# Autodesk Inventor assembly: Assembly1
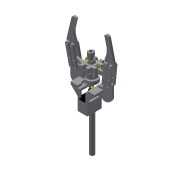
[picture p0: Inventor's stored thumbnail of the model, 180x180]
Saved by Autodesk Inventor 2018 (Build 220112000, 112)
## iProperties
Created: 2018-02-12
Part Number: Assembly1
Document SubType Name: Assembly
Designer: Bardo91
Author: Bardo91
## Documents named in this file (9)
- E:\programming\hecatonquiros\cad_models\tools\gripper\serial_model\Assembly1.iam
- E:\programming\hecatonquiros\cad_models\tools\gripper\serial_model\core_structure.ipt
- E:\programming\hecatonquiros\cad_models\tools\gripper\serial_model\holdBar.ipt
- E:\programming\hecatonquiros\cad_models\tools\gripper\serial_model\ScrewActuatorGripper.ipt
- E:\programming\hecatonquiros\cad_models\tools\gripper\serial_model\microservo_FT.ipt
- E:\programming\hecatonquiros\cad_models\tools\gripper\serial_model\bar.ipt
- E:\programming\hecatonquiros\cad_models\tools\gripper\serial_model\gripper.ipt
- E:\programming\hecatonquiros\cad_models\tools\gripper\serial_model\ScrewActuatorGripperCenter.ipt
- E:\programming\hecatonquiros\cad_models\tools\gripper\serial_model\barMini.ipt
## Components (18 placed, 8 different names)
1. core_structure:1 — Mate:1, Mate:2, Mate:3, Mate:4, Mate:5, Mate:6, Mate:7, Mate:8, Mate:9, Mate:10
2. holdBar:1 — Mate:4, Mate:5, Mate:6, Mate:11, Mate:12, Mate:13, Mate:14, Mate:15, Mate:16, Mate:17, Mate:18
3. holdBar:2 — Mate:1, Mate:2, Mate:3, Mate:19, Mate:20, Mate:21, Mate:22, Mate:23, Mate:24, Mate:25, Mate:26
4. ScrewActuatorGripper:1 — Mate:7, Mate:37, Mate:38
5. microservo_FT:1 — Mate:8, Mate:9, Mate:10
6. bar:1 — Mate:11, Mate:12, Mate:31
7. bar:2 — Mate:13, Mate:14, Mate:30, Mate:40
8. bar:3 — Mate:15, Mate:18, Mate:27, Mate:28
9. bar:4 — Mate:16, Mate:17, Mate:29
10. bar:5 — Mate:19, Mate:21, Mate:34, Mate:42
11. bar:6 — Mate:20, Mate:22, Mate:32, Mate:33
12. bar:7 — Mate:23, Mate:26, Mate:35
13. bar:8 — Mate:24, Mate:25, Mate:36
14. gripper:1 — Mate:27, Mate:28, Mate:29, Mate:30, Mate:31
15. gripper:2 — Mate:32, Mate:33, Mate:34, Mate:35, Mate:36
16. ScrewActuatorGripperCenter:1 — Mate:37, Mate:38, Mate:39, Mate:41, Mate:43, Mate:44
17. barMini:1 — Mate:39, Mate:40, Mate:41
18. barMini:2 — Mate:42, Mate:43, Mate:44
## Relationships (44: Mate 44)
- Mate:1: core_structure:1 ↔ holdBar:2
- Mate:2: core_structure:1 ↔ holdBar:2
- Mate:3: core_structure:1 ↔ holdBar:2
- Mate:4: core_structure:1 ↔ holdBar:1
- Mate:5: core_structure:1 ↔ holdBar:1
- Mate:6: core_structure:1 ↔ holdBar:1
- Mate:7: core_structure:1 ↔ ScrewActuatorGripper:1
- Mate:8: core_structure:1 ↔ microservo_FT:1
- Mate:9: core_structure:1 ↔ microservo_FT:1
- Mate:10: core_structure:1 ↔ microservo_FT:1
- Mate:11: holdBar:1 ↔ bar:1
- Mate:12: holdBar:1 ↔ bar:1
- Mate:13: holdBar:1 ↔ bar:2
- Mate:14: holdBar:1 ↔ bar:2
- Mate:15: holdBar:1 ↔ bar:3
- Mate:16: holdBar:1 ↔ bar:4
- Mate:17: holdBar:1 ↔ bar:4
- Mate:18: holdBar:1 ↔ bar:3
- Mate:19: holdBar:2 ↔ bar:5
- Mate:20: holdBar:2 ↔ bar:6
- Mate:21: holdBar:2 ↔ bar:5
- Mate:22: holdBar:2 ↔ bar:6
- Mate:23: holdBar:2 ↔ bar:7
- Mate:24: holdBar:2 ↔ bar:8
- Mate:25: holdBar:2 ↔ bar:8
- Mate:26: holdBar:2 ↔ bar:7
- Mate:27: bar:3 ↔ gripper:1
- Mate:28: bar:3 ↔ gripper:1
- Mate:29: bar:4 ↔ gripper:1
- Mate:30: bar:2 ↔ gripper:1
- Mate:31: bar:1 ↔ gripper:1
- Mate:32: bar:6 ↔ gripper:2
- Mate:33: bar:6 ↔ gripper:2
- Mate:34: bar:5 ↔ gripper:2
- Mate:35: bar:7 ↔ gripper:2
- Mate:36: bar:8 ↔ gripper:2
- Mate:37: ScrewActuatorGripper:1 ↔ ScrewActuatorGripperCenter:1
- Mate:38: ScrewActuatorGripper:1 ↔ ScrewActuatorGripperCenter:1
- Mate:39: ScrewActuatorGripperCenter:1 ↔ barMini:1
- Mate:40: bar:2 ↔ barMini:1
- Mate:41: ScrewActuatorGripperCenter:1 ↔ barMini:1
- Mate:42: bar:5 ↔ barMini:2
- Mate:43: ScrewActuatorGripperCenter:1 ↔ barMini:2
- Mate:44: ScrewActuatorGripperCenter:1 ↔ barMini:2
